# Autodesk Inventor assembly: robot
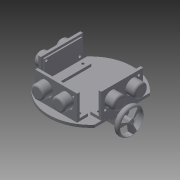
[picture p0: Inventor's stored thumbnail of the model, 180x180]
Saved by Autodesk Inventor 2015 (Build 190159000, 159)
## iProperties
Created: 2014-10-25
Part Number: robot
Document SubType Name: Assembly
Designer: Colin
Author: Colin
## Documents named in this file (4)
- E:\Users\Colin\Documents\college\marc\MicroMouse\robot.iam
- E:\Users\Colin\Documents\college\marc\MicroMouse\base.ipt
- E:\Users\Colin\Documents\college\marc\MicroMouse\wheel_assembly.iam
- E:\Users\Colin\Documents\college\marc\MicroMouse\ping_assembly.iam
## Components (6 placed, 3 different names)
1. base:1 — Flush:1, Flush:2, Mate:5, Mate:7, Mate:8, Mate:9, Mate:10, Flush:3, Mate:11, Flush:4, Mate:12, Mate:13, Flush:6, Mate:14
2. wheel_assembly:1 [sub-assembly] — Flush:1, Mate:5, Mate:8
3. wheel_assembly:2 [sub-assembly] — Flush:2, Mate:7, Mate:9
4. ping_assembly:1 [sub-assembly] — Flush:4, Mate:12, Flush:5
5. ping_assembly:2 [sub-assembly] — Mate:13, Flush:6, Mate:14
6. ping_assembly:3 [sub-assembly] — Mate:10, Flush:3, Mate:11, Flush:5
## Relationships (15: Mate 9, Flush 6)
- Flush:1: base:1 ↔ wheel_assembly:1
- Flush:2: base:1 ↔ wheel_assembly:2
- Mate:5: base:1 ↔ wheel_assembly:1
- Mate:7: base:1 ↔ wheel_assembly:2
- Mate:8 (46.9011 mm): base:1 ↔ wheel_assembly:1
- Mate:9 (20.3073 mm): base:1 ↔ wheel_assembly:2
- Mate:10: base:1 ↔ ping_assembly:3
- Flush:3: base:1 ↔ ping_assembly:3
- Mate:11 (8.0772 mm): base:1 ↔ ping_assembly:3
- Flush:4: base:1 ↔ ping_assembly:1
- Mate:12: base:1 ↔ ping_assembly:1
- Flush:5: ping_assembly:1 ↔ ping_assembly:3
- Mate:13: base:1 ↔ ping_assembly:2
- Flush:6 (12.7 mm): base:1 ↔ ping_assembly:2
- Mate:14 (-5.08 mm): base:1 ↔ ping_assembly:2
